# Autodesk Inventor assembly: Prototype II Assembly V3
(part 2 of 2)
- Mate:301: Union Elbow 1-8 KQ2L01-00A SMC:33 ↔ Cable Clip 3-1Dia RS817-8956:14
- Mate:302: Union Elbow 1-8 KQ2L01-00A SMC:33 ↔ Cable Clip 3-1Dia RS817-8956:14
- Mate:303: Union Elbow 1-8 KQ2L01-00A SMC:31 ↔ Cable Clip 3-1Dia RS817-8956:15
- Mate:304: Union Elbow 1-8 KQ2L01-00A SMC:31 ↔ Cable Clip 3-1Dia RS817-8956:15
- Mate:305: Union Elbow 1-8 KQ2L01-00A SMC:31 ↔ Cable Clip 3-1Dia RS817-8956:16
- Mate:306: Union Elbow 1-8 KQ2L01-00A SMC:31 ↔ Cable Clip 3-1Dia RS817-8956:16
- Mate:309: Union Elbow 1-8 KQ2L01-00A SMC:18 ↔ Cable Clip 3-1Dia RS817-8956:22
- Mate:310: Union Elbow 1-8 KQ2L01-00A SMC:18 ↔ Cable Clip 3-1Dia RS817-8956:22
- Mate:313: Internal Rear Plate:1 ↔ Union Tee 1-8 KQ2T01-00A SMC:1
- Mate:314: Internal Rear Plate:1 ↔ Union Elbow 1-8 KQ2L01-00A SMC:30
- Mate:315 (20 mm): Union Elbow 1-8 KQ2L01-00A SMC:17 ↔ Cable Clip 3-1Dia RS817-8956:25
- Mate:316: Union Elbow 1-8 KQ2L01-00A SMC:17 ↔ Cable Clip 3-1Dia RS817-8956:25
- Mate:318: Union Elbow 1-8 KQ2L01-00A SMC:21 ↔ Cable Clip 3-1Dia RS817-8956:24
- Mate:319: Union Elbow 1-8 KQ2L01-00A SMC:21 ↔ Cable Clip 3-1Dia RS817-8956:24
- Mate:322: Union Elbow 1-8 KQ2L01-00A SMC:1 ↔ Cable Clip 3-1Dia RS817-8956:19
- Mate:323: Union Elbow 1-8 KQ2L01-00A SMC:1 ↔ Cable Clip 3-1Dia RS817-8956:19
- Mate:324: Union Elbow 1-8 KQ2L01-00A SMC:30 ↔ Cable Clip 3-1Dia RS817-8956:26
- Mate:325: Union Elbow 1-8 KQ2L01-00A SMC:30 ↔ Cable Clip 3-1Dia RS817-8956:26
- Mate:326 (20 mm): Union Elbow 1-8 KQ2L01-00A SMC:29 ↔ Cable Clip 3-1Dia RS817-8956:27
- Mate:327: Union Elbow 1-8 KQ2L01-00A SMC:29 ↔ Cable Clip 3-1Dia RS817-8956:27
- Mate:328 (10 mm): Union Elbow 1-8 KQ2L01-00A SMC:23 ↔ Cable Clip 3-1Dia RS817-8956:20
- Mate:329: Union Elbow 1-8 KQ2L01-00A SMC:23 ↔ Cable Clip 3-1Dia RS817-8956:20
- Mate:330: Union Tee 1-8 KQ2T01-00A SMC:3 ↔ Cable Clip 3-1Dia RS817-8956:3
- Mate:332: Union Tee 1-8 KQ2T01-00A SMC:2 ↔ Cable Clip 3-1Dia RS817-8956:29
- Mate:333: Union Tee 1-8 KQ2T01-00A SMC:2 ↔ Cable Clip 3-1Dia RS817-8956:29
- Mate:334: Union Tee 1-8 KQ2T01-00A SMC:3 ↔ Cable Clip 3-1Dia RS817-8956:3
- Mate:337: Union Elbow 1-8 KQ2L01-00A SMC:2 ↔ Union Elbow 1-8 KQ2L01-00A SMC:11
- Mate:338: Union Elbow 1-8 KQ2L01-00A SMC:2 ↔ Cable Clip 3-1Dia RS817-8956:30
- Mate:339: Union Elbow 1-8 KQ2L01-00A SMC:2 ↔ Cable Clip 3-1Dia RS817-8956:30
- Mate:340: Internal Rear Plate:1 ↔ Valve Assembly:2
- Mate:341: Internal Rear Plate:1 ↔ Valve Assembly:3
- Mate:342: Internal Rear Plate:1 ↔ Valve Assembly:1
- Mate:343: Internal Rear Plate:1 ↔ Union Elbow 1-8 KQ2L01-00A SMC:31
- Mate:344: Internal Rear Plate:1 ↔ Switch Mode PS PCB:1
- Mate:345: SMC10-32UNF-1-8 KQ2H01-32N RS 840-4665:2 ↔ Union Elbow 1-8 KQ2L01-00A SMC:15
- Flush:29: Full Cartridge Interface:1 ↔ Control & Sense Head PCB Assm:1
- Mate:346 (0.8 mm): Full Cartridge Interface:1 ↔ Control & Sense Head PCB Assm:1
- Flush:30: Full Cartridge Interface:1 ↔ Control & Sense Head PCB Assm:1
- Mate:348: Internal Rear Plate:1 ↔ Union Elbow 1-8 KQ2L01-00A SMC:17
- Mate:349: Internal Rear Plate:1 ↔ Union Elbow 1-8 KQ2L01-00A SMC:23
- Mate:350: Internal Rear Plate:1 ↔ Union Elbow 1-8 KQ2L01-00A SMC:19
- Mate:352: Internal Rear Plate:1 ↔ Cable Clip 3-1Dia RS817-8956:20
- Mate:353: Internal Rear Plate:1 ↔ Union Tee 1-8 KQ2T01-00A SMC:1
- Mate:354: Internal Rear Plate:1 ↔ Union Elbow 1-8 KQ2L01-00A SMC:22
- Tangent:1 (94.05 mm): Enclosure RS746-7396 body:1 ↔ Door Lock:2
- Tangent:2 (29.25 mm): Enclosure RS746-7396 body:1 ↔ Door Lock:2
- Tangent:3 (29.25 mm): Enclosure RS746-7396 body:1 ↔ Door Lock:1
- Tangent:4 (274.05 mm): Enclosure RS746-7396 body:1 ↔ Door Lock:1
- Mate:364: Internal Rear Plate:1 ↔ Union Elbow 1-8 KQ2L01-00A SMC:29
- Angle:60 (0 deg): Internal Rear Plate:1 ↔ Union Elbow 1-8 KQ2L01-00A SMC:7
- Angle:61 (0 deg): Internal Rear Plate:1 ↔ Union Elbow 1-8 KQ2L01-00A SMC:30
- Angle:62 (0 deg): Internal Rear Plate:1 ↔ Union Elbow 1-8 KQ2L01-00A SMC:29
- Angle:63 (0 deg): Internal Rear Plate:1 ↔ Union Elbow 1-8 KQ2L01-00A SMC:17
- Angle:64 (0 deg): Internal Rear Plate:1 ↔ Union Tee 1-8 KQ2T01-00A SMC:2
- Mate:370: Union Elbow 1-8 KQ2L01-00A SMC:10 ↔ Union Tee 1-8 KQ2T01-00A SMC:2
- Angle:65 (0 deg): Internal Rear Plate:1 ↔ Union Elbow 1-8 KQ2L01-00A SMC:17
- Mate:371: 40ml Bottle and Lid:4 ↔ Union Elbow 1-8 KQ2L01-00A SMC:7
- Mate:372: Union Elbow 1-8 KQ2L01-00A SMC:8 ↔ Union Elbow 1-8 KQ2L01-00A SMC:30
- Flush:31 (60 mm): Port Support Plate:1 ↔ Mounted Pump:1
- Mate:374 (55 mm): Top Divider:1 ↔ Mounted Pump:1
- Mate:375 (10 mm): Mechanical Driver Board:1 ↔ Port Support Plate:1
- Mate:376: Top Divider:1 ↔ SMC AS2002F Needle Valve RS 827-0755:1
- Mate:377: Top Divider:1 ↔ SMC AS2002F Needle Valve RS 827-0755:1
- Mate:378: Mechanical Driver Board:1 ↔ Port Support Plate:1
- Mate:379: Mechanical Driver Board:1 ↔ Port Support Plate:1
- Mate:383: 22Ah BatteryPack:2 ↔ Internal Vert Divider:1
- Mate:384: Battery Base Plate:1 ↔ BAttery divider:1
- Mate:385 (0.025 mm): Battery Base Plate:1 ↔ BAttery divider:1
- Mate:386: Internal Rear Plate:1 ↔ BAttery divider:1
- Mate:387: Internal Vert Divider:1 ↔ No Thrd Right Support Farnell1466881:3
- Mate:388: Top Divider:1 ↔ Right Bracket 30mm RS749-1686:6
- Mate:389: Top Divider:1 ↔ Right Bracket 30mm RS749-1686:6
- Mate:390: Top Divider:1 ↔ Right Bracket 30mm RS749-1686:6
- Mate:391: Right Bracket 30mm RS749-1686:6 ↔ Internal Vert Divider:1
- Mate:392: Internal Rear Plate:1 ↔ Right Bracket 50mm RS749-1680:12
- Mate:393: Internal Rear Plate:1 ↔ Right Bracket 50mm RS749-1680:12
- Mate:394: Internal Rear Plate:1 ↔ Right Bracket 50mm RS749-1680:12
- Mate:395: Right Bracket 50mm RS749-1680:12 ↔ BAttery divider:1
- Mate:396: Right Bracket 50mm RS749-1680:12 ↔ BAttery divider:1
- Mate:397: Top Divider:1 ↔ Right Bracket 30mm RS749-1686:5
- Mate:398: Right Bracket 30mm RS749-1686:5 ↔ BAttery divider:1
- Mate:399: Top Divider:1 ↔ Right Bracket 30mm RS749-1686:5
- Mate:400: Right Bracket 30mm RS749-1686:5 ↔ BAttery divider:1
- Mate:401: Right Bracket 30mm RS749-1686:4 ↔ Battery Base Plate:1
- Mate:402: Right Bracket 30mm RS749-1686:4 ↔ BAttery divider:1
- Mate:403: Right Bracket 30mm RS749-1686:4 ↔ Battery Base Plate:1
- Mate:404: Right Bracket 30mm RS749-1686:3 ↔ Battery Side Plate:1
- Mate:405: Right Bracket 30mm RS749-1686:3 ↔ Battery Base Plate:1
- Mate:406: Right Bracket 30mm RS749-1686:3 ↔ Battery Side Plate:1
- Mate:407: Right Bracket 30mm RS749-1686:3 ↔ Battery Base Plate:1
- Mate:408: Right Bracket 30mm RS749-1686:2 ↔ Battery Base Plate:1
- Mate:409: Right Bracket 30mm RS749-1686:2 ↔ Internal Vert Divider:1
- Mate:410: Right Bracket 30mm RS749-1686:2 ↔ Internal Vert Divider:1
- Mate:411: Right Bracket 30mm RS749-1686:2 ↔ Battery Base Plate:1
- Mate:412: Internal Rear Plate:1 ↔ Right Bracket 30mm RS749-1686:9
- Mate:413: Internal Vert Divider:1 ↔ Right Bracket 30mm RS749-1686:9
- Mate:414: Internal Rear Plate:1 ↔ Right Bracket 30mm RS749-1686:9
- Mate:415 (0.5 mm): 22Ah BatteryPack:1 ↔ Battery Con:2
- Angle:66 (0 deg): Battery Con:2 ↔ BAttery divider:1
- Mate:416: 22Ah BatteryPack:1 ↔ Battery Con:2
- Mate:417: 22Ah BatteryPack:1 ↔ Battery Con:2
- Mate:418: Top Divider:1 ↔ Right Bracket 30mm RS749-1686:10
- Mate:419: Battery Side Plate:1 ↔ Right Bracket 30mm RS749-1686:10
- Mate:420: Battery Side Plate:1 ↔ Right Bracket 30mm RS749-1686:10
- Mate:421: Top Divider:1 ↔ Right Bracket 30mm RS749-1686:10
- Mate:422: Bottle Base Plate:1 ↔ No Thrd Right Support Farnell1466881:9
- Mate:423: Internal Rear Plate:1 ↔ Bottle side plate:1
- Mate:424: Bottle Base Plate:1 ↔ Bottle side plate:1
- Flush:32: Bottle Base Plate:1 ↔ Bottle side plate:1
- Mate:446: Internal Rear Plate:1 ↔ No Thrd Right Support Farnell1466881:6
- Mate:447: No Thrd Right Support Farnell1466881:5 ↔ Bottle side plate:1
- Mate:448: No Thrd Right Support Farnell1466881:4 ↔ Bottle side plate:1
- Mate:449: Internal Rear Plate:1 ↔ No Thrd Right Support Farnell1466881:6
- Mate:450: Bottle Base Plate:1 ↔ No Thrd Right Support Farnell1466881:6
- Mate:451: Bottle Base Plate:1 ↔ No Thrd Right Support Farnell1466881:6
- Mate:452: No Thrd Right Support Farnell1466881:5 ↔ Bottle side plate:1
- Mate:453: Bottle Base Plate:1 ↔ No Thrd Right Support Farnell1466881:5
- Mate:454: Bottle Base Plate:1 ↔ No Thrd Right Support Farnell1466881:4
- Mate:455: No Thrd Right Support Farnell1466881:4 ↔ Bottle side plate:1
- Mate:456: Bottle Base Plate:1 ↔ No Thrd Right Support Farnell1466881:5
- Mate:457: Bottle Base Plate:1 ↔ No Thrd Right Support Farnell1466881:4
- Mate:458: Bottle Base Plate:1 ↔ No Thrd Right Support Farnell1466881:9
- Mate:459: Internal Vert Divider:1 ↔ No Thrd Right Support Farnell1466881:9
- Mate:460: Bottle Base Plate:1 ↔ No Thrd Right Support Farnell1466881:13
- Mate:461: Internal Vert Divider:1 ↔ No Thrd Right Support Farnell1466881:13
- Mate:462: Internal Vert Divider:1 ↔ No Thrd Right Support Farnell1466881:13
- Mate:463: Bottle Base Plate:1 ↔ No Thrd Right Support Farnell1466881:13
- Mate:464: Battery Side Plate:1 ↔ Battery Top Plate:1
- Mate:465: Internal Rear Plate:1 ↔ Battery Top Plate:1
- Mate:466: BAttery divider:1 ↔ Battery Top Plate:1
- Mate:467: Internal Rear Plate:1 ↔ No Thrd Right Support Farnell1466881:12
- Mate:468: Internal Rear Plate:1 ↔ No Thrd Right Support Farnell1466881:7
- Mate:469: Internal Rear Plate:1 ↔ No Thrd Right Support Farnell1466881:11
- Mate:470: Internal Rear Plate:1 ↔ No Thrd Right Support Farnell1466881:8
- Mate:471: Battery Side Plate:1 ↔ No Thrd Right Support Farnell1466881:19
- Mate:472: Battery Top Plate:1 ↔ No Thrd Right Support Farnell1466881:20
- Mate:473: Battery Top Plate:1 ↔ No Thrd Right Support Farnell1466881:18
- Mate:474: Battery Top Plate:1 ↔ No Thrd Right Support Farnell1466881:17
- Mate:475: Battery Top Plate:1 ↔ No Thrd Right Support Farnell1466881:21
- Mate:476: Battery Top Plate:1 ↔ No Thrd Right Support Farnell1466881:16
- Mate:477: Battery Top Plate:1 ↔ No Thrd Right Support Farnell1466881:19
- Mate:478: No Thrd Right Support Farnell1466881:11 ↔ Battery Top Plate:1
- Mate:479: No Thrd Right Support Farnell1466881:8 ↔ Battery Top Plate:1
- Mate:480: BAttery divider:1 ↔ No Thrd Right Support Farnell1466881:20
- Mate:481: BAttery divider:1 ↔ No Thrd Right Support Farnell1466881:18
- Mate:482: Battery Top Plate:1 ↔ No Thrd Right Support Farnell1466881:18
- Mate:483: Battery Top Plate:1 ↔ No Thrd Right Support Farnell1466881:20
- Mate:484: BAttery divider:1 ↔ No Thrd Right Support Farnell1466881:20
- Mate:485: No Thrd Right Support Farnell1466881:8 ↔ Battery Top Plate:1
- Mate:486: Internal Rear Plate:1 ↔ No Thrd Right Support Farnell1466881:8
- Mate:487: Internal Rear Plate:1 ↔ No Thrd Right Support Farnell1466881:11
- Mate:488: No Thrd Right Support Farnell1466881:11 ↔ Battery Top Plate:1
- Mate:489: Battery Top Plate:1 ↔ No Thrd Right Support Farnell1466881:19
- Mate:490: Battery Side Plate:1 ↔ No Thrd Right Support Farnell1466881:19
- Mate:491: BAttery divider:1 ↔ No Thrd Right Support Farnell1466881:18
- Mate:492: Battery Top Plate:1 ↔ No Thrd Right Support Farnell1466881:17
- Mate:493: BAttery divider:1 ↔ No Thrd Right Support Farnell1466881:17
- Mate:494: BAttery divider:1 ↔ No Thrd Right Support Farnell1466881:17
- Mate:495: No Thrd Right Support Farnell1466881:12 ↔ Battery Top Plate:1
- Mate:496: No Thrd Right Support Farnell1466881:7 ↔ Battery Top Plate:1
- Mate:497: Internal Vert Divider:1 ↔ No Thrd Right Support Farnell1466881:21
- Mate:498: Internal Vert Divider:1 ↔ No Thrd Right Support Farnell1466881:16
- Mate:499: No Thrd Right Support Farnell1466881:12 ↔ Battery Top Plate:1
- Mate:500: Internal Rear Plate:1 ↔ No Thrd Right Support Farnell1466881:12
- Mate:501: No Thrd Right Support Farnell1466881:7 ↔ Battery Top Plate:1
- Mate:502: Internal Rear Plate:1 ↔ No Thrd Right Support Farnell1466881:7
- Mate:503: Battery Top Plate:1 ↔ No Thrd Right Support Farnell1466881:21
- Mate:504: Battery Top Plate:1 ↔ No Thrd Right Support Farnell1466881:16
- Mate:505: Internal Vert Divider:1 ↔ No Thrd Right Support Farnell1466881:16
- Mate:506: Internal Vert Divider:1 ↔ No Thrd Right Support Farnell1466881:21
- Mate:507: Internal Rear Plate:1 ↔ Right Bracket 50mm RS749-1680:15
- Mate:508: Right Bracket 50mm RS749-1680:15 ↔ Bottle side plate:1
- Mate:509: Right Bracket 50mm RS749-1680:15 ↔ Bottle side plate:1
- Mate:510: Right Bracket 50mm RS749-1680:15 ↔ Bottle side plate:1
- Mate:511: Internal Rear Plate:1 ↔ Right Bracket 50mm RS749-1680:15
- Angle:67 (0 deg): Box Fixing Stud:3 ↔ Bottle Base Plate:1
- Mate:512: Internal Rear Plate:1 ↔ BS 4320 Form AB M8 (Form B):1
- Mate:513: Box Fixing Stud:3 ↔ BS 4320 Form AB M8 (Form B):1
- Mate:514: Box Fixing Stud:3 ↔ DIN 934 - replaced by DIN EN 24032/28673/28674 M8:2
- Mate:515: BS 4320 Form AB M8 (Form B):1 ↔ DIN 934 - replaced by DIN EN 24032/28673/28674 M8:2
- Mate:516: Internal Rear Plate:1 ↔ BS 4320 Form AB M8 (Form B):2
- Mate:517: Box Fixing Stud:2 ↔ BS 4320 Form AB M8 (Form B):2
- Mate:518: Internal Rear Plate:1 ↔ BS 4320 Form AB M8 (Form B):4
- Mate:519: Box Fixing Stud:4 ↔ BS 4320 Form AB M8 (Form B):4
- Mate:520: Internal Rear Plate:1 ↔ BS 4320 Form AB M8 (Form B):3
- Mate:521: Box Fixing Stud:1 ↔ BS 4320 Form AB M8 (Form B):3
- Mate:522: BS 4320 Form AB M8 (Form B):3 ↔ DIN 934 - replaced by DIN EN 24032/28673/28674 M8:3
- Mate:523: BS 4320 Form AB M8 (Form B):4 ↔ DIN 934 - replaced by DIN EN 24032/28673/28674 M8:4
- Mate:524: BS 4320 Form AB M8 (Form B):2 ↔ DIN 934 - replaced by DIN EN 24032/28673/28674 M8:1
- Mate:525: Box Fixing Stud:2 ↔ DIN 934 - replaced by DIN EN 24032/28673/28674 M8:1
- Mate:526: Box Fixing Stud:4 ↔ DIN 934 - replaced by DIN EN 24032/28673/28674 M8:4
- Mate:527: Box Fixing Stud:1 ↔ DIN 934 - replaced by DIN EN 24032/28673/28674 M8:3
- Mate:528: Internal Rear Plate:1 ↔ Bottle Spacer Base:1
- Mate:529: Internal Vert Divider:1 ↔ Bottle Spacer Base:1
- Mate:530 (16 mm): Bottle Base Plate:1 ↔ Bottle Spacer Base:1
- Mate:531: Internal Vert Divider:1 ↔ Lower slide:2
- Mate:532: Bottle Base Plate:1 ↔ Lower slide:2
- Mate:533: Internal Vert Divider:1 ↔ Lower slide:2
- Mate:535: Bottle Base Plate:1 ↔ Lower slide:1
- Mate:536: Bottle side plate:1 ↔ Lower slide:1
- Mate:537: Bottle side plate:1 ↔ Lower slide:1
- Mate:538: Bottle side plate:1 ↔ Lower slide:1
- Mate:539: Internal Vert Divider:1 ↔ Upper slide:2
- Mate:540: Internal Vert Divider:1 ↔ Upper slide:2
- Mate:541: Internal Vert Divider:1 ↔ Upper slide:2
- Mate:542: Bottle side plate:1 ↔ Upper slide:1
- Mate:543: Bottle side plate:1 ↔ Upper slide:1
- Mate:544: Bottle side plate:1 ↔ Upper slide:1
- Mate:545: Bottle side plate:1 ↔ Single Thrd Right Support Farnell1466883:13
- Mate:546: Bottle side plate:1 ↔ Single Thrd Right Support Farnell1466883:13
- Angle:68 (180 deg): Single Thrd Right Support Farnell1466883:13 ↔ Bottle Spacer Base:1
- Mate:547: Single Thrd Right Support Farnell1466883:13 ↔ Bottle Spacer Base:1
- Mate:548: Internal Vert Divider:1 ↔ Single Thrd Right Support Farnell1466883:9
- Mate:549: Internal Vert Divider:1 ↔ Single Thrd Right Support Farnell1466883:9
- Angle:69 (180 deg): Single Thrd Right Support Farnell1466883:9 ↔ Bottle Spacer Base:1
- Mate:550: Single Thrd Right Support Farnell1466883:9 ↔ Bottle Spacer Base:1
- Mate:551: Top Divider:1 ↔ Gas Side Top Cover:1
- Mate:552: Bottle side plate:1 ↔ Gas Side Top Cover:1
- Flush:33: Top Divider:1 ↔ Gas Side Top Cover:1
- Flush:34: Top Divider:1 ↔ Battery Cover:1
- Flush:35: Internal Vert Divider:1 ↔ Battery Cover:1
- Mate:553: Top Divider:1 ↔ Battery Cover:1
- Mate:554: Top Divider:1 ↔ Electronics cover:1
- Mate:556: Top Divider:1 ↔ Single Thrd Right Support Farnell1466883:15
- Mate:557: Top Divider:1 ↔ Single Thrd Right Support Farnell1466883:10
- Mate:558: Battery Side Plate:1 ↔ Single Thrd Right Support Farnell1466883:16
- Mate:559: Single Thrd Right Support Farnell1466883:17 ↔ Battery Top Plate:1
- Mate:560: Single Thrd Right Support Farnell1466883:18 ↔ Battery Top Plate:1
- Mate:561: Internal Vert Divider:1 ↔ Single Thrd Right Support Farnell1466883:19
- Mate:562: Internal Vert Divider:1 ↔ Single Thrd Right Support Farnell1466883:25
- Mate:563: BAttery divider:1 ↔ Single Thrd Right Support Farnell1466883:20
- Mate:564: Battery Base Plate:1 ↔ Single Thrd Right Support Farnell1466883:21
- Mate:565: Battery Base Plate:1 ↔ Single Thrd Right Support Farnell1466883:8
- Mate:566: Battery Base Plate:1 ↔ Single Thrd Right Support Farnell1466883:26
- Mate:567: Battery Base Plate:1 ↔ Single Thrd Right Support Farnell1466883:22
- Mate:568: BAttery divider:1 ↔ Single Thrd Right Support Farnell1466883:20
- Mate:569: Battery Base Plate:1 ↔ Single Thrd Right Support Farnell1466883:26
- Mate:570: Battery Base Plate:1 ↔ Single Thrd Right Support Farnell1466883:22
- Mate:571: Battery Base Plate:1 ↔ Single Thrd Right Support Farnell1466883:8
- Mate:572: Battery Base Plate:1 ↔ Single Thrd Right Support Farnell1466883:21
- Mate:573: Internal Vert Divider:1 ↔ Single Thrd Right Support Farnell1466883:25
- Flush:36: Internal Vert Divider:1 ↔ Single Thrd Right Support Farnell1466883:25
- Flush:37: Battery Base Plate:1 ↔ Single Thrd Right Support Farnell1466883:21
- Flush:38: Battery Base Plate:1 ↔ Single Thrd Right Support Farnell1466883:8
- Flush:39: Battery Base Plate:1 ↔ Single Thrd Right Support Farnell1466883:26
- Flush:40: Battery Base Plate:1 ↔ Single Thrd Right Support Farnell1466883:22
- Flush:41: BAttery divider:1 ↔ Single Thrd Right Support Farnell1466883:20
- Mate:574: Battery Side Plate:1 ↔ Single Thrd Right Support Farnell1466883:32
- Mate:575: Battery Side Plate:1 ↔ Single Thrd Right Support Farnell1466883:32
- Flush:42: Battery Side Plate:1 ↔ Single Thrd Right Support Farnell1466883:32
- Mate:576: Single Thrd Right Support Farnell1466883:18 ↔ Battery Top Plate:1
- Mate:577: Internal Vert Divider:1 ↔ Single Thrd Right Support Farnell1466883:19
- Mate:578: Single Thrd Right Support Farnell1466883:17 ↔ Battery Top Plate:1
- Mate:579: Battery Side Plate:1 ↔ Single Thrd Right Support Farnell1466883:16
- Mate:580: Top Divider:1 ↔ Single Thrd Right Support Farnell1466883:10
- Mate:581: Top Divider:1 ↔ Single Thrd Right Support Farnell1466883:15
- Flush:43: Single Thrd Right Support Farnell1466883:18 ↔ Battery Top Plate:1
- Flush:44: Single Thrd Right Support Farnell1466883:17 ↔ Battery Top Plate:1
- Angle:70 (180 deg): Single Thrd Right Support Farnell1466883:19 ↔ Battery Top Plate:1
- Flush:45: Top Divider:1 ↔ Single Thrd Right Support Farnell1466883:15
- Flush:46: Top Divider:1 ↔ Single Thrd Right Support Farnell1466883:10
- Flush:47: Battery Side Plate:1 ↔ Single Thrd Right Support Farnell1466883:16
- Mate:582: Bottle side plate:1 ↔ Single Thrd Right Support Farnell1466883:27
- Mate:583: Top Divider:1 ↔ Single Thrd Right Support Farnell1466883:28
- Mate:584: Top Divider:1 ↔ Single Thrd Right Support Farnell1466883:29
- Mate:585: Internal Vert Divider:1 ↔ Single Thrd Right Support Farnell1466883:31
- Mate:586: Internal Vert Divider:1 ↔ Single Thrd Right Support Farnell1466883:23
- Mate:587: Internal Vert Divider:1 ↔ Single Thrd Right Support Farnell1466883:24
- Mate:588: Internal Vert Divider:1 ↔ Single Thrd Right Support Farnell1466883:24
- Mate:589: Internal Vert Divider:1 ↔ Single Thrd Right Support Farnell1466883:23
- Mate:590: Internal Vert Divider:1 ↔ Single Thrd Right Support Farnell1466883:31
- Mate:591: Top Divider:1 ↔ Single Thrd Right Support Farnell1466883:29
- Mate:592: Top Divider:1 ↔ Single Thrd Right Support Farnell1466883:28
- Mate:593: Bottle side plate:1 ↔ Single Thrd Right Support Farnell1466883:27
- Angle:71 (0 deg): Bottle side plate:1 ↔ Single Thrd Right Support Farnell1466883:27
- Angle:72 (0 deg): Top Divider:1 ↔ Single Thrd Right Support Farnell1466883:28
- Angle:73 (0 deg): Top Divider:1 ↔ Single Thrd Right Support Farnell1466883:29
- Angle:74 (180 deg): Top Divider:1 ↔ Single Thrd Right Support Farnell1466883:31
- Angle:75 (0 deg): Top Divider:1 ↔ Single Thrd Right Support Farnell1466883:23
- Angle:76 (0 deg): Single Thrd Right Support Farnell1466883:23 ↔ Single Thrd Right Support Farnell1466883:24
- Mate:594: Top Divider:1 ↔ Single Thrd Right Support Farnell1466883:33
- Mate:595: Top Divider:1 ↔ Single Thrd Right Support Farnell1466883:34
- Mate:596: Top Divider:1 ↔ Single Thrd Right Support Farnell1466883:36
- Mate:598: Inner Top Plate:1 ↔ Single Thrd Right Support Farnell1466883:37
- Mate:599: Inner Top Plate:1 ↔ Single Thrd Right Support Farnell1466883:35
- Mate:603: Top Divider:1 ↔ Single Thrd Right Support Farnell1466883:33
- Mate:604: Top Divider:1 ↔ Single Thrd Right Support Farnell1466883:34
- Mate:605: Top Divider:1 ↔ Single Thrd Right Support Farnell1466883:36
- Angle:77 (0 deg): Top Divider:1 ↔ Single Thrd Right Support Farnell1466883:36
- Angle:78 (0 deg): Top Divider:1 ↔ Single Thrd Right Support Farnell1466883:34
- Angle:79 (0 deg): Top Divider:1 ↔ Single Thrd Right Support Farnell1466883:33
- Mate:607: Internal Rear Plate:1 ↔ corner spacers:4
- Mate:608: Fixing Stud Pt 2:1 ↔ corner spacers:4
- Mate:609: Internal Rear Plate:1 ↔ corner spacers:3
- Mate:610: Box Fixing Stud:2 ↔ corner spacers:3
- Mate:611: Internal Rear Plate:1 ↔ corner spacers:2
- Mate:612: Box Fixing Stud:3 ↔ corner spacers:2
- Angle:80 (0 deg): Internal Rear Plate:1 ↔ corner spacers:2
- Mate:613: Internal Rear Plate:1 ↔ corner spacers:1
- Mate:614: Box Fixing Stud:1 ↔ corner spacers:1
- Angle:81 (0 deg): Internal Rear Plate:1 ↔ corner spacers:1
- Mate:615: Box Fixing Stud:2 ↔ Silicone Seal washer:3
- Mate:616: Box Fixing Stud:3 ↔ Silicone Seal washer:4
- Mate:617: Fixing Stud Pt 2:3 ↔ Silicone Seal washer:3
- Mate:618: Fixing Stud Pt 2:2 ↔ Silicone Seal washer:4
- Mate:619: Box Fixing Stud:4 ↔ Silicone Seal washer:2
- Mate:620: Fixing Stud Pt 2:1 ↔ Silicone Seal washer:2
- Mate:621: Fixing Stud Pt 2:4 ↔ Silicone Seal washer:1
- Mate:622: 22Ah BatteryPack:2 ↔ Battery Con:1
- Mate:623: Inner Top Plate:1 ↔ Single Thrd Right Support Farnell1466883:41
- Mate:624: Inner Top Plate:1 ↔ Single Thrd Right Support Farnell1466883:41
- Mate:625: Inner Top Plate:1 ↔ Single Thrd Right Support Farnell1466883:38
- Mate:626: Inner Top Plate:1 ↔ Single Thrd Right Support Farnell1466883:38
- Mate:627: Inner Top Plate:1 ↔ Single Thrd Right Support Farnell1466883:40
- Mate:629: Coms Board V1:1 ↔ Single Thrd Right Support Farnell1466883:41
- Mate:630: Coms Board V1:1 ↔ Single Thrd Right Support Farnell1466883:38
- Mate:631: Coms Board V1:1 ↔ Single Thrd Right Support Farnell1466883:41
- Mate:632: Top Divider:1 ↔ Single Thrd Right Support Farnell1466883:39
- Mate:633: Top Divider:1 ↔ Single Thrd Right Support Farnell1466883:39
- Mate:634: Top Divider:1 ↔ Single Thrd Right Support Farnell1466883:42
- Mate:635: Top Divider:1 ↔ Single Thrd Right Support Farnell1466883:42
- Mate:636: Coms Board V1:1 ↔ Single Thrd Right Support Farnell1466883:39
- Mate:637: Coms Board V1:1 ↔ Single Thrd Right Support Farnell1466883:42
- Mate:638: Electronics cover:1 ↔ Single Thrd Right Support Farnell1466883:33
- Mate:639: Electronics cover:1 ↔ Single Thrd Right Support Farnell1466883:33
- Mate:640: Electronics cover:1 ↔ Step-back spacer -electronics enc:1
- Mate:641: Electronics cover:1 ↔ Step-back spacer -electronics enc:1
- Mate:642: Electronics cover:1 ↔ Step-back spacer -electronics enc:1
- Mate:643: Step-back spacer -electronics enc:1 ↔ Step-back cover -electronics enc:1
- Mate:644: Step-back spacer -electronics enc:1 ↔ Step-back cover -electronics enc:1
- Mate:645: Step-back spacer -electronics enc:1 ↔ Step-back cover -electronics enc:1
- Mate:646: Upper slide:1 ↔ Top Bottle Back:1
- Mate:647: Internal Vert Divider:1 ↔ Top Bottle Back:1
- Mate:648: Internal Rear Plate:1 ↔ Top Bottle Back:1
- Mate:649: Upper slide:2 ↔ Top Bottle Middle:1
- Mate:650: Bottle side plate:1 ↔ Top Bottle Middle:1
- Mate:651: Top Bottle Middle:1 ↔ Top Bottle Back:1
- Mate:652: Upper slide:2 ↔ Top Bottle Front:1
- Mate:653: Top Bottle Front:1 ↔ Top Bottle Middle:1
- Mate:654: Bottle side plate:1 ↔ Top Bottle Front:1
- Mate:655: Upper slide:1 ↔ Single Thrd Right Support Farnell1466883:43
- Mate:656: Upper slide:2 ↔ Single Thrd Right Support Farnell1466883:44
- Mate:657: Upper slide:2 ↔ Single Thrd Right Support Farnell1466883:44
- Mate:658: Upper slide:1 ↔ Single Thrd Right Support Farnell1466883:43
- Angle:82 (180 deg): Top Bottle Front:1 ↔ Single Thrd Right Support Farnell1466883:43
- Angle:83 (180 deg): Top Bottle Front:1 ↔ Single Thrd Right Support Farnell1466883:44
- Mate:659: Bottle side plate:1 ↔ upper plate slide:1
- Mate:660: Top Bottle Middle:1 ↔ upper plate slide:1
- Mate:661: Internal Rear Plate:1 ↔ upper plate slide:1
- Mate:662: Internal Vert Divider:1 ↔ upper plate slide:2
- Mate:663: Top Bottle Middle:1 ↔ upper plate slide:2
- Mate:664: Internal Rear Plate:1 ↔ upper plate slide:2
- Mate:665: Internal Vert Divider:1 ↔ upper plate slide:2
- Mate:666: Internal Vert Divider:1 ↔ upper plate slide:2
- Mate:667: Inner Top Plate:1 ↔ Single Thrd Right Support Farnell1466883:35
- Mate:668: Inner Top Plate:1 ↔ Single Thrd Right Support Farnell1466883:40
- Mate:669: Inner Top Plate:1 ↔ Single Thrd Right Support Farnell1466883:37
- Mate:670 (5 mm): Status Indicator PCB:1 ↔ Inner Top Plate:1
- Mate:671: Status Indicator PCB:1 ↔ Inner Top Plate:1
- Mate:672: Status Indicator PCB:1 ↔ Inner Top Plate:1
- Mate:673 (7 mm): Top Divider:1 ↔ LiPo cover:1
- Mate:675: Coms Board V1:1 ↔ Single Thrd Right Support Farnell1466883:39
- Mate:676: Top Divider:1 ↔ Lipo Battery:1
- Flush:48 (7.5 mm): LiPo cover:1 ↔ Lipo Battery:1
- Mate:677: Internal Vert Divider:1 ↔ Lower slide:2
- Mate:678: Top Divider:1 ↔ LipoBat Spacer:2
- Mate:679: Top Divider:1 ↔ LipoBat Spacer:1
- Mate:680: Top Divider:1 ↔ LipoBat Spacer:1
- Mate:681: Top Divider:1 ↔ LipoBat Spacer:1
- Mate:682 (62 mm): LipoBat Spacer:1 ↔ LipoBat Spacer:2
- Flush:50: LipoBat Spacer:1 ↔ LipoBat Spacer:2
